# Autodesk Inventor assembly: untitled.brd
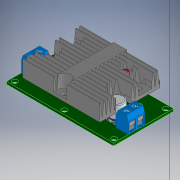
[picture p0: Inventor's stored thumbnail of the model, 180x180]
Saved by Autodesk Inventor 2022 (Build 260153000, 153)
## iProperties
Created: 2022-12-24
Part Number: untitled.brd
Document SubType Name: Assembly
Designer: Ivan Petrov
Author: Ivan Petrov
## Documents named in this file (9)
- C:\Users\Ivan Petrov\Documents\GitHub\OmniBot\design\000.007 - Бортовой источник питания СБ.iam
- C:\Users\Ivan Petrov\Documents\GitHub\OmniBot\design\000.007.001 - Плата печатная.ipt
- C:\Users\Ivan Petrov\Documents\GitHub\OmniBot\design\standart_components\TO-PMOD NDY-11.ipt
- C:\Users\Ivan Petrov\Documents\GitHub\OmniBot\design\standart_components\smd resistors\0R.iam
- C:\Users\Ivan Petrov\Documents\GitHub\OmniBot\design\standart_components\Capacitors smd\Сборка1.iam
- C:\Users\Ivan Petrov\Documents\GitHub\OmniBot\design\standart_components\Capacitors smd\05_NICHICON_8X10_NEWARK_58R3566_ENSAMBLE.ipt
- C:\Users\Ivan Petrov\Documents\GitHub\OmniBot\design\standart_components\LED-Red.ipt
- C:\Users\Ivan Petrov\Documents\GitHub\OmniBot\design\standart_components\Capacitors smd\000.007.002 - Радиатор.ipt
- C:\Users\Ivan Petrov\Documents\GitHub\OmniBot\design\standart_components\Terminal Block 2P.ipt
## Components (22 placed, 20 different names)
1. untitled.brdКонтур:1 — Совмещение:2, Совмещение:11, Совмещение:20, Совмещение:21, Совмещение:22, Совмещение:23, Совмещение:24, Совмещение:25, Угол:1, Совмещение:26, Угол:2
2. C1_2 [sub-assembly]
3. C2_3 [sub-assembly]
4. C3_4 [sub-assembly]
5. C4_5 [sub-assembly]
6. C5_6 [sub-assembly]
7. C6_7 [sub-assembly]
8. C7_8 [sub-assembly]
9. C8_9 [sub-assembly]
10. R1_24 [sub-assembly]
11. R2_25 [sub-assembly]
12. R3_26 [sub-assembly]
13. R4_27 [sub-assembly]
14. R5_28 [sub-assembly]
15. R6_29 [sub-assembly]
16. TO-PMOD NDY-11:1 — Совмещение:2, Заподлицо:1, Совмещение:27
17. 05_NICHICON_8X10_NEWARK_58R3566_ENSAMBLE:1 — Совмещение:10, Совмещение:11
18. 05_NICHICON_8X10_NEWARK_58R3566_ENSAMBLE:2 — Совмещение:19, Совмещение:20
19. LED-Red:1 — Совмещение:21, Совмещение:22, Заподлицо:1
20. 000.007.002 - Радиатор:1 — Совмещение:27
21. Terminal Block 2P:1 — Совмещение:23, Совмещение:25, Угол:1
22. Terminal Block 2P:2 — Совмещение:24, Совмещение:26, Угол:2
## Relationships (21: Mate 18, Angle 2, Flush 1)
- Совмещение:2 [Mate]: untitled.brdКонтур:1 ↔ TO-PMOD NDY-11:1
- Совмещение:7 [Mate]
- Совмещение:8 [Mate]
- Совмещение:9 [Mate]
- Совмещение:10 [Mate]: 05_NICHICON_8X10_NEWARK_58R3566_ENSAMBLE:1
- Совмещение:11 [Mate]: untitled.brdКонтур:1 ↔ 05_NICHICON_8X10_NEWARK_58R3566_ENSAMBLE:1
- Совмещение:16 [Mate]
- Совмещение:17 [Mate]
- Совмещение:18 [Mate]
- Совмещение:19 [Mate]: 05_NICHICON_8X10_NEWARK_58R3566_ENSAMBLE:2
- Совмещение:20 [Mate]: untitled.brdКонтур:1 ↔ 05_NICHICON_8X10_NEWARK_58R3566_ENSAMBLE:2
- Совмещение:21 [Mate]: untitled.brdКонтур:1 ↔ LED-Red:1
- Совмещение:22 [Mate]: untitled.brdКонтур:1 ↔ LED-Red:1
- Заподлицо:1 [Flush]: TO-PMOD NDY-11:1 ↔ LED-Red:1
- Совмещение:23 [Mate]: untitled.brdКонтур:1 ↔ Terminal Block 2P:1
- Совмещение:24 [Mate]: untitled.brdКонтур:1 ↔ Terminal Block 2P:2
- Совмещение:25 [Mate]: untitled.brdКонтур:1 ↔ Terminal Block 2P:1
- Угол:1 [Angle] (-90 deg): untitled.brdКонтур:1 ↔ Terminal Block 2P:1
- Совмещение:26 [Mate]: untitled.brdКонтур:1 ↔ Terminal Block 2P:2
- Угол:2 [Angle] (0 deg): untitled.brdКонтур:1 ↔ Terminal Block 2P:2
- Совмещение:27 [Mate]: TO-PMOD NDY-11:1 ↔ 000.007.002 - Радиатор:1
